# Autodesk Inventor assembly: DATN
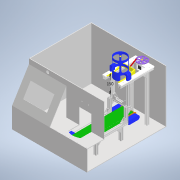
[picture p0: Inventor's stored thumbnail of the model, 180x180]
Saved by Autodesk Inventor 2020 (Build 240168000, 168)
## iProperties
Created: 2022-12-11
Part Number: DATN
Document SubType Name: Assembly
Designer: ADMIN
Author: ADMIN
## Documents named in this file (3)
- D:\Do-an-tot-nghiep\Inventor\DATN.iam
- D:\Do-an-tot-nghiep\Inventor\Vỏ máy.iam
- D:\Do-an-tot-nghiep\Inventor\Khung máy.iam
## Components (2 placed, 2 different names)
1. Vỏ máy:1 [sub-assembly] — Mate:1, Flush:1
2. Khung máy:2 [sub-assembly] — Mate:1, Flush:2
## Relationships (3: Flush 2, Mate 1)
- Mate:1: Vỏ máy:1 ↔ Khung máy:2
- Flush:1 (-150 mm): Vỏ máy:1
- Flush:2 (-80 mm): Khung máy:2
